# Autodesk Inventor assembly: A101EnsembleChariot
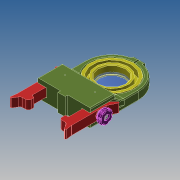
[picture p0: Inventor's stored thumbnail of the model, 180x180]
Saved by Autodesk Inventor 2017 (Build 210142000, 142)
## iProperties
Created: 2016-10-17
Part Number: A101EnsembleChariot
Document SubType Name: Assembly
Designer: serge.amoos
Author: serge.amoos
## Documents named in this file (13)
- I:\RaD\SI-ET\Projets\51346-SmartLens\inventor\FocalMeasure\A101EnsembleChariot.iam
- I:\RaD\SI-ET\Projets\51346-SmartLens\inventor\FocalMeasure\p102chariotArrondi.ipt
- I:\RaD\SI-ET\Projets\51346-SmartLens\inventor\FocalMeasure\P103Bielle.ipt
- I:\RaD\SI-ET\Projets\51346-SmartLens\inventor\FocalMeasure\p104levier1.ipt
- I:\RaD\SI-ET\Projets\51346-SmartLens\inventor\FocalMeasure\p105levier2.ipt
- I:\RaD\SI-ET\Projets\51346-SmartLens\inventor\FocalMeasure\P109Ecrou.ipt
- I:\RaD\SI-ET\Projets\51346-SmartLens\inventor\FocalMeasure\P110Poussoir.ipt
- I:\RaD\SI-ET\Projets\51346-SmartLens\inventor\FocalMeasure\F105ViTcyl6pcM3x12.ipt
- I:\RaD\SI-ET\Projets\51346-SmartLens\inventor\FocalMeasure\P111Molette.ipt
- I:\RaD\SI-ET\Projets\51346-SmartLens\inventor\FocalMeasure\F106EcrouM3.ipt
- I:\RaD\SI-ET\Projets\51346-SmartLens\inventor\FocalMeasure\P113TigeFileteeM3.ipt
- I:\RaD\SI-ET\Projets\51346-SmartLens\inventor\FocalMeasure\p118portelentille30mm.ipt
- I:\RaD\SI-ET\Projets\51346-SmartLens\inventor\FocalMeasure\F117Lens30mm.ipt
## Components (15 placed, 12 different names)
1. p102chariotArrondi:1 — Mate:1, Mate:2, Flush:1, Angle:1, Mate:4, Mate:5, Mate:6, Insert:1, Insert:2, Insert:3, Insert:4, Angle:2, Flush:2, Flush:3, Insert:7
2. P103Bielle:1 — Mate:1, Mate:2, Mate:3
3. p104levier1:1 — Flush:1, Mate:3, Angle:1, Mate:10, Tangent:1, Flush:2
4. P103Bielle:2 — Mate:4, Mate:5, Mate:7
5. P109Ecrou:1 — Mate:8, Mate:9
6. p105levier2:1 — Mate:6, Mate:7, Mate:8, Mate:9, Flush:3
7. P110Poussoir:1 — Insert:2
8. P110Poussoir:2 — Insert:1
9. F105ViTcyl6pcM3x12:1 — Insert:3
10. P111Molette:1 — Mate:10, Tangent:1, Insert:6, Mate:11, Mate:12, Flush:4
11. F106EcrouM3:1 — Insert:4, Angle:2
12. P113TigeFileteeM3:1 — Mate:12, Flush:4
13. F106EcrouM3:2 — Insert:6, Mate:11
14. p118portelentille30mm:1 — Insert:7, Insert:8
15. F117Lens30mm:1 — Insert:8
## Relationships (26: Mate 12, Insert 7, Flush 4, Angle 2, Tangent 1)
- Mate:1: p102chariotArrondi:1 ↔ P103Bielle:1
- Mate:2: p102chariotArrondi:1 ↔ P103Bielle:1
- Flush:1: p102chariotArrondi:1 ↔ p104levier1:1
- Mate:3: P103Bielle:1 ↔ p104levier1:1
- Angle:1 (0 deg): p102chariotArrondi:1 ↔ p104levier1:1
- Mate:4: p102chariotArrondi:1 ↔ P103Bielle:2
- Mate:5: p102chariotArrondi:1 ↔ P103Bielle:2
- Mate:6: p102chariotArrondi:1 ↔ p105levier2:1
- Mate:7: P103Bielle:2 ↔ p105levier2:1
- Mate:8: P109Ecrou:1 ↔ p105levier2:1
- Mate:9: P109Ecrou:1 ↔ p105levier2:1
- Insert:1: p102chariotArrondi:1 ↔ P110Poussoir:2
- Insert:2: p102chariotArrondi:1 ↔ P110Poussoir:1
- Mate:10: p104levier1:1 ↔ P111Molette:1
- Tangent:1: p104levier1:1 ↔ P111Molette:1
- Insert:3: p102chariotArrondi:1 ↔ F105ViTcyl6pcM3x12:1
- Insert:4: p102chariotArrondi:1 ↔ F106EcrouM3:1
- Angle:2 (0 deg): p102chariotArrondi:1 ↔ F106EcrouM3:1
- Insert:6: P111Molette:1 ↔ F106EcrouM3:2
- Mate:11: P111Molette:1 ↔ F106EcrouM3:2
- Flush:2 (1 mm): p102chariotArrondi:1 ↔ p104levier1:1
- Flush:3 (-1 mm): p102chariotArrondi:1 ↔ p105levier2:1
- Mate:12: P111Molette:1 ↔ P113TigeFileteeM3:1
- Flush:4: P111Molette:1 ↔ P113TigeFileteeM3:1
- Insert:7: p102chariotArrondi:1 ↔ p118portelentille30mm:1
- Insert:8: p118portelentille30mm:1 ↔ F117Lens30mm:1
